# Autodesk Inventor assembly: COROA(43) - PINHÃO(54)
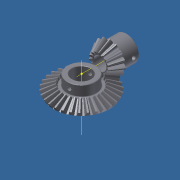
[picture p0: Inventor's stored thumbnail of the model, 180x180]
Saved by Autodesk Inventor 2012 SP2 (Build 160219200, 219)
## iProperties
Created: 2012-07-24
Part Number: COROA(43) - PINHÃO(54)
Document SubType Name: Assembly
Designer: bruno.silveira
Author: bruno.silveira
## Documents named in this file (2)
- H:\CAD\BASSOTTI\Documents\DESENHOS.CAD-BRUNOBASSOTTI\DESENHOS-AUTODESK-INVENTOR\CAMINHÃO-BITONEIRA-(SENAI)\COROA(43) - PINHÃO(54)\COROA(43) - PINHÃO(54).iam
- H:\CAD\BASSOTTI\Documents\DESENHOS.CAD-BRUNOBASSOTTI\DESENHOS-AUTODESK-INVENTOR\CAMINHÃO-BITONEIRA-(SENAI)\COROA(43) - PINHÃO(54)\Design Accelerator\Bevel Gears1.iam
## Components (1 placed, 1 different names)
1. Bevel Gears:1 [sub-assembly] — Mate:9, Angle:3, Mate:10, Angle:4, Angle:5
## Relationships (17: Mate 10, Angle 5, Flush 2)
- Flush:1 (20 mm)
- Flush:2 (17 mm)
- Mate:1
- Mate:2
- Mate:3
- Mate:4
- Mate:5
- Angle:1 (90 deg)
- Mate:6
- Angle:2 (0 deg)
- Mate:7
- Mate:8
- Mate:9: Bevel Gears:1
- Angle:3 (0 deg): Bevel Gears:1
- Mate:10: Bevel Gears:1
- Angle:4 (0 deg): Bevel Gears:1
- Angle:5 (0 deg): Bevel Gears:1
